# Autodesk Inventor assembly: JewlArm
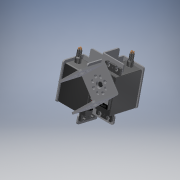
[picture p0: Inventor's stored thumbnail of the model, 180x180]
Saved by Autodesk Inventor 2017 (Build 210142000, 142)
## iProperties
Created: 2017-10-12
Part Number: JewlArm
Document SubType Name: Assembly
Designer: User
Author: User
## Documents named in this file (4)
- C:\Robotics\CAD\2017-18_CAD\Miscellaneous\JewlArm.iam
- C:\Robotics\CAD\COTSParts\Tetrix\Tetrix servo 180.ipt
- C:\Robotics\CAD\COTSParts\Tetrix\Tetrix bracket - single servo.ipt
- C:\Robotics\CAD\COTSParts\Tetrix\Tetrix channel 32mm.ipt
## Components (5 placed, 3 different names)
1. Tetrix servo 180:1 — Insert:7, Mate:4, Mate:11, Mate:12, Mate:13
2. Tetrix servo 180:2 — Mate:9, Mate:10, Mate:15, Mate:16, Mate:17
3. Tetrix bracket - single servo:1 — Mate:15, Mate:16, Mate:17
4. Tetrix bracket - single servo:2 — Mate:9, Mate:10, Mate:11, Mate:12, Mate:13
5. Tetrix channel 32mm:1 — Insert:7, Mate:4
## Relationships (10: Mate 9, Insert 1)
- Insert:7: Tetrix servo 180:1 ↔ Tetrix channel 32mm:1
- Mate:4: Tetrix servo 180:1 ↔ Tetrix channel 32mm:1
- Mate:9: Tetrix servo 180:2 ↔ Tetrix bracket - single servo:2
- Mate:10: Tetrix servo 180:2 ↔ Tetrix bracket - single servo:2
- Mate:11: Tetrix servo 180:1 ↔ Tetrix bracket - single servo:2
- Mate:12: Tetrix servo 180:1 ↔ Tetrix bracket - single servo:2
- Mate:13: Tetrix servo 180:1 ↔ Tetrix bracket - single servo:2
- Mate:15: Tetrix servo 180:2 ↔ Tetrix bracket - single servo:1
- Mate:16: Tetrix servo 180:2 ↔ Tetrix bracket - single servo:1
- Mate:17: Tetrix servo 180:2 ↔ Tetrix bracket - single servo:1
